# Autodesk Inventor assembly: Сборка1
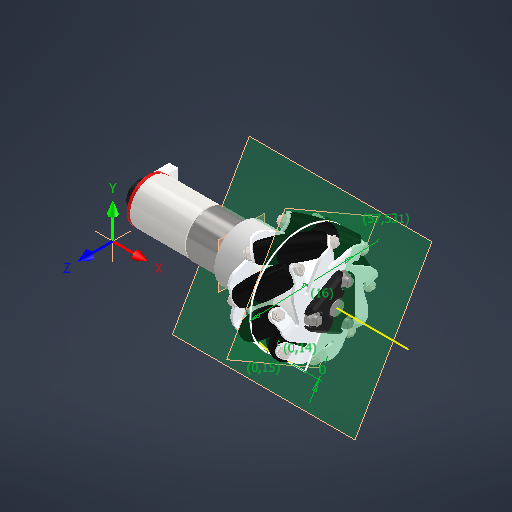
[picture p0: Inventor's stored thumbnail of the model, 512x512]
Saved by Autodesk Inventor 2025 (Build 290162000, 162)
## iProperties
Created: 2024-12-25
Part Number: Сборка1
Document SubType Name: Assembly
Designer: khrip
Author: khrip
## Documents named in this file (4)
- H:\Potamon\3Dmodels\SusUnit\Сборка1.iam
- H:\Potamon\3Dmodels\UnsprungUnits\Wheels\wheel assembly.iam
- H:\Potamon\3Dmodels\UnsprungUnits\Parts\servo.ipt
- H:\Potamon\3Dmodels\UnsprungUnits\Parts\Knuckle.ipt
## Components (3 placed, 3 different names)
1. wheel assembly:1 [sub-assembly]
2. servo:1
3. Knuckle:1
## Relationships (4: Mate 2, Flush 2)
- [Mate]: wheel assembly:1 ↔ servo:1
- [Mate] (0.5 mm): wheel assembly:1 ↔ servo:1
- [Flush]: wheel assembly:1 ↔ Knuckle:1
- [Flush]: servo:1 ↔ Knuckle:1
